# Autodesk Inventor assembly: VDPiller_B
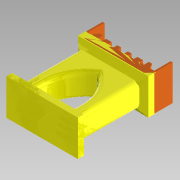
[picture p0: Inventor's stored thumbnail of the model, 180x180]
Saved by Autodesk Inventor 2021 (Build 250183000, 183)
## iProperties
Created: 2021-03-10
Part Number: VDPiller_B
Document SubType Name: Assembly
Designer: kumagai
Author: kumagai
## Documents named in this file (3)
- X:\Develop\CAD\PlaRails\ViaductPillar\VDPillar_B.iam
- X:\Develop\CAD\PlaRails\ViaductPillar\PillarTopVD.ipt
- X:\Develop\CAD\PlaRails\ViaductPillar\VDPillar_B.ipt
## Components (2 placed, 2 different names)
1. PillarTopVD:1
2. VDPillar_B:1 — フラッシュ:1, フラッシュ:4, フラッシュ:5
## Relationships (3: Flush 3)
- フラッシュ:1 [Flush]: VDPillar_B:1
- フラッシュ:4 [Flush]: VDPillar_B:1
- フラッシュ:5 [Flush]: VDPillar_B:1
